# Autodesk Inventor assembly: Redesign_GripperASSEM
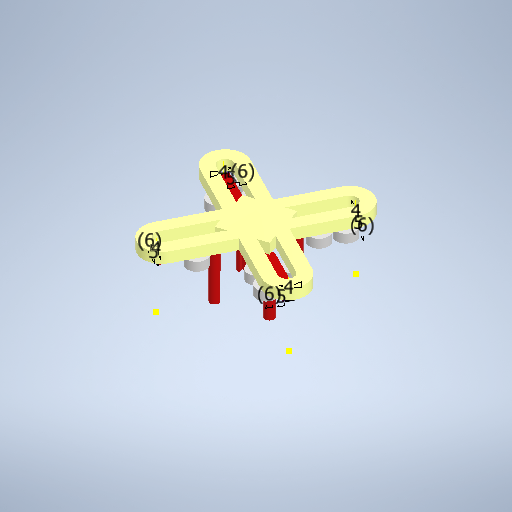
[picture p0: Inventor's stored thumbnail of the model, 512x512]
Saved by Autodesk Inventor 2025.1 (Build 291241000, 241)
## iProperties
Created: 2024-12-20
Part Number: Redesign_GripperASSEM
Document SubType Name: Assembly
Designer: m_kni
Author: m_kni
## Documents named in this file (4)
- C:\Users\m_kni\OneDrive\Documents\GitHub\Perovskite-Automated-Synthesis-System\CAD\Gripper\Redesign_GripperASSEM.iam
- C:\Users\m_kni\OneDrive\Documents\GitHub\Perovskite-Automated-Synthesis-System\CAD\Gripper\Redesign_Gripper_Baseplate.ipt
- C:\Users\m_kni\OneDrive\Documents\GitHub\Perovskite-Automated-Synthesis-System\CAD\Gripper\5x5x11bearing.ipt
- C:\Users\m_kni\OneDrive\Documents\GitHub\Perovskite-Automated-Synthesis-System\CAD\Gripper\Redesign_Gripper_Finger.ipt
## Components (17 placed, 3 different names)
1. Redesign_Gripper_Baseplate:1 — Insert:1, Insert:2, Insert:3, Insert:4, Insert:5, Insert:6, Insert:7, Insert:8, Insert:9, Insert:10, Insert:11, Insert:12, Mate:3, Mate:4, Mate:6, Mate:8
2. 5x5x11bearing:1 — Insert:7, Tangent:3
3. 5x5x11bearing:2 — Insert:8, Tangent:8
4. 5x5x11bearing:3 — Insert:5, Tangent:4
5. 5x5x11bearing:4 — Insert:1, Tangent:5, Mate:5
6. 5x5x11bearing:5 — Insert:2
7. 5x5x11bearing:6 — Insert:3, Tangent:7, Mate:7
8. 5x5x11bearing:7 — Insert:4
9. 5x5x11bearing:8 — Insert:10, Tangent:1
10. 5x5x11bearing:9 — Insert:6, Mate:2
11. 5x5x11bearing:10 — Insert:12, Mate:1
12. 5x5x11bearing:11 — Insert:11, Tangent:2
13. 5x5x11bearing:12 — Insert:9, Tangent:6
14. Redesign_Gripper_Finger:1 — Tangent:1, Tangent:2, Mate:1, Mate:4
15. Redesign_Gripper_Finger:2 — Tangent:3, Mate:2, Tangent:4, Mate:3
16. Redesign_Gripper_Finger:3 — Tangent:5, Tangent:6, Mate:5, Mate:6
17. Redesign_Gripper_Finger:4 — Tangent:7, Tangent:8, Mate:7, Mate:8
## Relationships (28: Insert 12, Tangent 8, Mate 8)
- Insert:1: Redesign_Gripper_Baseplate:1 ↔ 5x5x11bearing:4
- Insert:2: Redesign_Gripper_Baseplate:1 ↔ 5x5x11bearing:5
- Insert:3: Redesign_Gripper_Baseplate:1 ↔ 5x5x11bearing:6
- Insert:4: Redesign_Gripper_Baseplate:1 ↔ 5x5x11bearing:7
- Insert:5: Redesign_Gripper_Baseplate:1 ↔ 5x5x11bearing:3
- Insert:6: Redesign_Gripper_Baseplate:1 ↔ 5x5x11bearing:9
- Insert:7: Redesign_Gripper_Baseplate:1 ↔ 5x5x11bearing:1
- Insert:8: Redesign_Gripper_Baseplate:1 ↔ 5x5x11bearing:2
- Insert:9: Redesign_Gripper_Baseplate:1 ↔ 5x5x11bearing:12
- Insert:10: Redesign_Gripper_Baseplate:1 ↔ 5x5x11bearing:8
- Insert:11: Redesign_Gripper_Baseplate:1 ↔ 5x5x11bearing:11
- Insert:12: Redesign_Gripper_Baseplate:1 ↔ 5x5x11bearing:10
- Tangent:1: 5x5x11bearing:8 ↔ Redesign_Gripper_Finger:1
- Tangent:2: 5x5x11bearing:11 ↔ Redesign_Gripper_Finger:1
- Mate:1: 5x5x11bearing:10 ↔ Redesign_Gripper_Finger:1
- Tangent:3: 5x5x11bearing:1 ↔ Redesign_Gripper_Finger:2
- Mate:2: 5x5x11bearing:9 ↔ Redesign_Gripper_Finger:2
- Tangent:4: 5x5x11bearing:3 ↔ Redesign_Gripper_Finger:2
- Mate:3: Redesign_Gripper_Baseplate:1 ↔ Redesign_Gripper_Finger:2
- Mate:4: Redesign_Gripper_Baseplate:1 ↔ Redesign_Gripper_Finger:1
- Tangent:5: 5x5x11bearing:4 ↔ Redesign_Gripper_Finger:3
- Tangent:6: 5x5x11bearing:12 ↔ Redesign_Gripper_Finger:3
- Mate:5: 5x5x11bearing:4 ↔ Redesign_Gripper_Finger:3
- Mate:6: Redesign_Gripper_Baseplate:1 ↔ Redesign_Gripper_Finger:3
- Tangent:7: 5x5x11bearing:6 ↔ Redesign_Gripper_Finger:4
- Tangent:8: 5x5x11bearing:2 ↔ Redesign_Gripper_Finger:4
- Mate:7: 5x5x11bearing:6 ↔ Redesign_Gripper_Finger:4
- Mate:8: Redesign_Gripper_Baseplate:1 ↔ Redesign_Gripper_Finger:4
